# Autodesk Inventor assembly: FelAlvaz
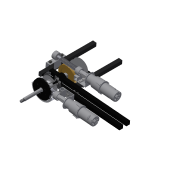
[picture p0: Inventor's stored thumbnail of the model, 180x180]
Saved by Autodesk Inventor 2015 SP1 (Build 190203100, 203)
## iProperties
Created: 2015-02-23
Part Number: FelAlvaz
Document SubType Name: Assembly
Designer: laca
Author: laca
## Documents named in this file (13)
- C:\Users\laca\Desktop\Allamvizsga\Invntor\RobotMechanikaForMAtlabVer2\FelAlvaz.iam
- C:\Users\laca\Desktop\Allamvizsga\Invntor\RobotMechanikaForMAtlabVer2\CsapágyHáz.ipt
- C:\Users\laca\Desktop\Allamvizsga\Invntor\RobotMechanikaForMAtlabVer2\EgyvégenMartSzelvény.ipt
- C:\Users\laca\Desktop\Allamvizsga\Invntor\RobotMechanikaForMAtlabVer2\KétvégenMartSzelvény.ipt
- C:\Users\laca\Desktop\Allamvizsga\Invntor\RobotMechanikaForMAtlabVer2\6001 BEARING.iam
- C:\Users\laca\Desktop\Allamvizsga\Invntor\RobotMechanikaForMAtlabVer2\ProvedoSenzor.iam
- C:\Users\laca\Desktop\Allamvizsga\Invntor\RobotMechanikaForMAtlabVer2\Talp.iam
- C:\Users\laca\Desktop\Allamvizsga\Invntor\RobotMechanikaForMAtlabVer2\KozepsoOsszekotok.ipt
- C:\Users\laca\Desktop\Allamvizsga\Invntor\RobotMechanikaForMAtlabVer2\SzéleségiSzelvény.ipt
- C:\Users\laca\Desktop\Allamvizsga\Invntor\RobotMechanikaForMAtlabVer2\InkrementalisFoliaEsNullAtmenet.iam
- C:\Users\laca\Desktop\Allamvizsga\Invntor\RobotMechanikaForMAtlabVer2\FelAlvaz\Design Accelerator\Bolted Connection1.iam
- C:\Users\laca\Desktop\Allamvizsga\Invntor\RobotMechanikaForMAtlabVer2\FelAlvaz\Design Accelerator\Bolted Connection5.iam
- C:\Users\laca\Desktop\Allamvizsga\Invntor\RobotMechanikaForMAtlabVer2\FelAlvaz\Design Accelerator\Bolted Connection2.iam
## Components (15 placed, 10 different names)
1. CsapágyHáz:1
2. EgyvégenMartSzelvény:1
3. KétvégenMartSzelvény:1 — Flush:14
4. EgyvégenMartSzelvény:3 — Rigid:11
5. KétvégenMartSzelvény:2 — Flush:3
6. 6001 BEARING:2 [sub-assembly]
7. 6001 BEARING:4 [sub-assembly] — Insert:7
8. ProvedoSenzor:1 [sub-assembly] — Insert:13
9. Talp:1 [sub-assembly] — Insert:7, Flush:3, Flush:8, Flush:9, Flush:12, Insert:13, Rigid:18, Mate:22, Mate:23, Mate:26, Mate:27, Mate:28, Mate:29
10. KozepsoOsszekotok:1 — Mate:2, Flush:12, Flush:13, Flush:14, Mate:30, Mate:31
11. SzéleségiSzelvény:1 — Rigid:11, Mate:2, Flush:8, Flush:9, Flush:13
12. InkrementalisFoliaEsNullAtmenet:1 [sub-assembly] — Rigid:18, Mate:30, Mate:31
13. Bolted Connection:1 [sub-assembly] — Mate:28, Mate:29
14. Bolted Connection:3 [sub-assembly] — Mate:22, Mate:23
15. Bolted Connection:4 [sub-assembly] — Mate:26, Mate:27
## Relationships (30: Mate 12, Flush 7, WeldJoint 6, Insert 5)
- [WeldJoint]: CsapágyHáz:1 ↔ KétvégenMartSzelvény:2
- [WeldJoint]: CsapágyHáz:1 ↔ KétvégenMartSzelvény:1
- [WeldJoint]: CsapágyHáz:1 ↔ EgyvégenMartSzelvény:1
- [WeldJoint]: CsapágyHáz:1 ↔ EgyvégenMartSzelvény:3
- [Insert]: CsapágyHáz:1 ↔ 6001 BEARING:2
- [Insert]: CsapágyHáz:1 ↔ 6001 BEARING:4
- [Insert]: CsapágyHáz:1 ↔ ProvedoSenzor:1
- [Flush]: KétvégenMartSzelvény:2 ↔ ProvedoSenzor:1
- Insert:7: 6001 BEARING:4 ↔ Talp:1
- Flush:3: KétvégenMartSzelvény:2 ↔ Talp:1
- Rigid:11 [WeldJoint]: EgyvégenMartSzelvény:3 ↔ SzéleségiSzelvény:1
- Mate:2 (97.5 mm): KozepsoOsszekotok:1 ↔ SzéleségiSzelvény:1
- Flush:8 (-2 mm): Talp:1 ↔ SzéleségiSzelvény:1
- Flush:9: Talp:1 ↔ SzéleségiSzelvény:1
- Mate:14
- Mate:15
- Mate:17
- Flush:12: Talp:1 ↔ KozepsoOsszekotok:1
- Insert:13: ProvedoSenzor:1 ↔ Talp:1
- Rigid:18 [WeldJoint]: Talp:1 ↔ InkrementalisFoliaEsNullAtmenet:1
- Mate:22: Talp:1 ↔ Bolted Connection:3
- Mate:23: Talp:1 ↔ Bolted Connection:3
- Flush:13: KozepsoOsszekotok:1 ↔ SzéleségiSzelvény:1
- Flush:14: KétvégenMartSzelvény:1 ↔ KozepsoOsszekotok:1
- Mate:26: Talp:1 ↔ Bolted Connection:4
- Mate:27: Talp:1 ↔ Bolted Connection:4
- Mate:28: Talp:1 ↔ Bolted Connection:1
- Mate:29: Talp:1 ↔ Bolted Connection:1
- Mate:30: KozepsoOsszekotok:1 ↔ InkrementalisFoliaEsNullAtmenet:1
- Mate:31: KozepsoOsszekotok:1 ↔ InkrementalisFoliaEsNullAtmenet:1
## Named parameters: d14_d18 = 0 mm, d16_d20 = 0 mm
